# Autodesk Inventor assembly: Assembly1
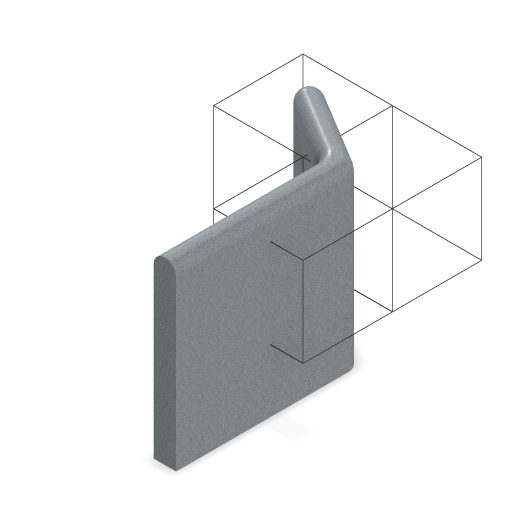
[picture p0: Inventor's stored thumbnail of the model, 512x512]
Saved by Autodesk Inventor 2023 (Build 270158000, 158)
## iProperties
Created: 2022-08-07
Part Number: Assembly1
Document SubType Name: Assembly
Designer: Derm
Author: Derm
## Documents named in this file (10)
- C:\Users\Derm\vaRLnt\v3\demo\sigmaPoint\Assembly1.iam
- C:\Users\Derm\vaRLnt\v3\demo\sigmaPoint\ellipse1.ipt
- C:\Users\Derm\vaRLnt\v3\demo\sigmaPoint\column.ipt
- C:\Users\Derm\vaRLnt\v3\demo\sigmaPoint\redPoint.ipt
- C:\Users\Derm\vaRLnt\v3\demo\sigmaPoint\voxel.ipt
- C:\Users\Derm\vaRLnt\v3\demo\sigmaPoint\smallerVoxel.ipt
- C:\Users\Derm\vaRLnt\v3\demo\sigmaPoint\ellipse2.ipt
- C:\Users\Derm\vaRLnt\v3\demo\sigmaPoint\ellipse3.ipt
- C:\Users\Derm\vaRLnt\v3\demo\sigmaPoint\ellipse4.ipt
- C:\Users\Derm\vaRLnt\v3\demo\sigmaPoint\wall.ipt
## Components (43 placed, 9 different names)
1. ellipse1:1
2. column:1
3. redPoint:1
4. voxel:1 — Mate:2
5. redPoint:2
6. redPoint:3
7. redPoint:4
8. redPoint:5
9. redPoint:6
10. redPoint:7
11. redPoint:8
12. redPoint:9
13. redPoint:10
14. redPoint:11
15. redPoint:12
16. redPoint:13
17. redPoint:14
18. redPoint:15
19. redPoint:16
20. redPoint:17
21. redPoint:18
22. redPoint:20
23. redPoint:21
24. redPoint:22
25. redPoint:23
26. redPoint:24
27. redPoint:25
28. redPoint:26
29. redPoint:27
30. redPoint:28
31. redPoint:29
32. redPoint:30
33. redPoint:31
34. smallerVoxel:1
35. ellipse2:1
36. ellipse3:1
37. ellipse4:1
38. ellipse1:2
39. voxel:2
40. wall:1
41. smallerVoxel:2 — Mate:3, Mate:4
42. smallerVoxel:3 — Mate:3, Mate:4, Mate:5, Mate:6
43. smallerVoxel:4 — Mate:5, Mate:6
## Relationships (5: Mate 5)
- Mate:2: voxel:1
- Mate:3: smallerVoxel:2 ↔ smallerVoxel:3
- Mate:4: smallerVoxel:2 ↔ smallerVoxel:3
- Mate:5: smallerVoxel:3 ↔ smallerVoxel:4
- Mate:6: smallerVoxel:3 ↔ smallerVoxel:4
